# Autodesk Inventor assembly: draftEndEffectorV2
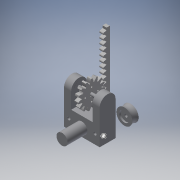
[picture p0: Inventor's stored thumbnail of the model, 180x180]
Saved by Autodesk Inventor 2017 (Build 210142000, 142)
## iProperties
Created: 2018-10-17
Part Number: draftEndEffectorV2
Document SubType Name: Assembly
Designer: Tom
Author: Tom
## Documents named in this file (7)
- C:\Users\Tom\Google Drive\UQ\UNI_WORK\METR4202\Problem Sets\PS3\CAD\draftEndEffectorV2.iam
- C:\Users\Tom\Google Drive\UQ\UNI_WORK\METR4202\Problem Sets\PS3\CAD\EndEffectorV2.ipt
- C:\Users\Tom\Google Drive\UQ\UNI_WORK\METR4202\Problem Sets\PS3\CAD\Pinion.ipt
- C:\Users\Tom\Google Drive\UQ\UNI_WORK\METR4202\Problem Sets\PS3\CAD\Rack.ipt
- C:\Users\Tom\Google Drive\UQ\UNI_WORK\METR4202\Problem Sets\PS3\CAD\shaft.ipt
- C:\Users\Tom\Google Drive\UQ\UNI_WORK\METR4202\Problem Sets\PS3\CAD\U-Groove-Bearings.ipt
- C:\Users\Tom\Google Drive\UQ\UNI_WORK\METR4202\Problem Sets\PS3\CAD\bearing.ipt
## Components (10 placed, 5 different names)
1. EndEffectorV2:1 — Mate:7, Flush:5, Mate:8, Mate:9, Mate:10, Angle:1
2. Spur Gear1:1 — Mate:5, Mate:6, Flush:6
3. Spur Gear1:2 — Flush:6
4. shaft:1 — Mate:3, Flush:1, Mate:4, Flush:2, Mate:5, Mate:7
5. U-Groove-Bearings:1 — Mate:1, Flush:3
6. U-Groove-Bearings:2 — Mate:2, Flush:4, Angle:1
7. bearing:1 — Mate:4, Flush:2, Mate:6, Flush:5
8. bearing:2 — Mate:3, Flush:1
9. bearing:3 — Mate:2, Flush:4, Mate:8, Mate:10
10. bearing:4 — Mate:1, Flush:3, Mate:9
## Relationships (17: Mate 10, Flush 6, Angle 1)
- Mate:1: U-Groove-Bearings:1 ↔ bearing:4
- Mate:2: U-Groove-Bearings:2 ↔ bearing:3
- Mate:3: shaft:1 ↔ bearing:2
- Flush:1: shaft:1 ↔ bearing:2
- Mate:4: shaft:1 ↔ bearing:1
- Flush:2: shaft:1 ↔ bearing:1
- Flush:3 (1 mm): U-Groove-Bearings:1 ↔ bearing:4
- Flush:4 (1 mm): U-Groove-Bearings:2 ↔ bearing:3
- Mate:5: Spur Gear1:1 ↔ shaft:1
- Mate:6 (11 mm): Spur Gear1:1 ↔ bearing:1
- Mate:7: EndEffectorV2:1 ↔ shaft:1
- Flush:5: EndEffectorV2:1 ↔ bearing:1
- Flush:6: Spur Gear1:1 ↔ Spur Gear1:2
- Mate:8: EndEffectorV2:1 ↔ bearing:3
- Mate:9: EndEffectorV2:1 ↔ bearing:4
- Mate:10: EndEffectorV2:1 ↔ bearing:3
- Angle:1 (180 deg): EndEffectorV2:1 ↔ U-Groove-Bearings:2
